# Autodesk Inventor assembly: rocket_asm
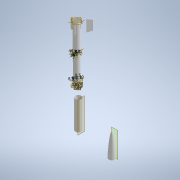
[picture p0: Inventor's stored thumbnail of the model, 180x180]
Saved by Autodesk Inventor 2020 (Build 240168000, 168)
## iProperties
Created: 2022-06-15
Part Number: rocket_asm
Document SubType Name: Assembly
Designer: sp
Author: sp
## Documents named in this file (12)
- C:\Users\sp\Desktop\neu_Rocket\rocket_asm.iam
- C:\Users\sp\Desktop\neu_Rocket\Engine.ipt
- C:\Users\sp\Desktop\neu_Rocket\Segment_elektro.ipt
- C:\Users\sp\Desktop\neu_Rocket\Segment_Engine.ipt
- C:\Users\sp\Desktop\neu_Rocket\Segment_recovery.ipt
- C:\Users\sp\Desktop\neu_Rocket\Spitze.ipt
- C:\Users\sp\Desktop\neu_Rocket\Leitwerk.ipt
- C:\Users\sp\Desktop\neu_Rocket\Back_holder.ipt
- C:\Users\sp\Desktop\neu_Rocket\Ronde_Engine.ipt
- C:\Users\sp\Desktop\neu_Rocket\recovery_asm.iam
- C:\Users\sp\Desktop\neu_Rocket\servo_asm.iam
- C:\Users\sp\Desktop\neu_Rocket\Deckel_Parachute_6.ipt
## Components (13 placed, 11 different names)
1. Engine:1 — Passend:1, Einfügen:1, Einfügen:2, Passend:2, Einfügen:3
2. Segment_elektro:1
3. Segment_Engine:1 — Einfügen:2, Passend:3, Passend:4, Passend:5, Passend:6, Passend:7, Passend:8, Einfügen:4
4. Segment_recovery:1 — Einfügen:5, Fluchtend:1, Einfügen:6
5. Spitze:1
6. Leitwerk:1 — Passend:7, Passend:8
7. Leitwerk:2 — Passend:3, Passend:4
8. Leitwerk:3 — Passend:5, Passend:6
9. Back_holder:1 — Passend:2, Einfügen:3
10. Ronde_Engine:1 — Passend:1, Einfügen:1
11. recovery_asm:1 [sub-assembly] — Einfügen:4, Einfügen:5, Fluchtend:1, Einfügen:7
12. servo_asm:1 [sub-assembly] — Einfügen:6
13. Deckel_Parachute_6:1 — Einfügen:7
## Relationships (16: Mate 8, Insert 7, Flush 1)
- Passend:1 [Mate]: Engine:1 ↔ Ronde_Engine:1
- Einfügen:1 [Insert]: Engine:1 ↔ Ronde_Engine:1
- Einfügen:2 [Insert]: Engine:1 ↔ Segment_Engine:1
- Passend:2 [Mate]: Engine:1 ↔ Back_holder:1
- Einfügen:3 [Insert]: Engine:1 ↔ Back_holder:1
- Passend:3 [Mate]: Segment_Engine:1 ↔ Leitwerk:2
- Passend:4 [Mate]: Segment_Engine:1 ↔ Leitwerk:2
- Passend:5 [Mate]: Segment_Engine:1 ↔ Leitwerk:3
- Passend:6 [Mate]: Segment_Engine:1 ↔ Leitwerk:3
- Passend:7 [Mate]: Segment_Engine:1 ↔ Leitwerk:1
- Passend:8 [Mate]: Segment_Engine:1 ↔ Leitwerk:1
- Einfügen:4 [Insert]: Segment_Engine:1 ↔ recovery_asm:1
- Einfügen:5 [Insert]: Segment_recovery:1 ↔ recovery_asm:1
- Fluchtend:1 [Flush]: Segment_recovery:1 ↔ recovery_asm:1
- Einfügen:6 [Insert]: Segment_recovery:1 ↔ servo_asm:1
- Einfügen:7 [Insert] (-73 mm): recovery_asm:1 ↔ Deckel_Parachute_6:1
